# Autodesk Inventor assembly: Ensemble1
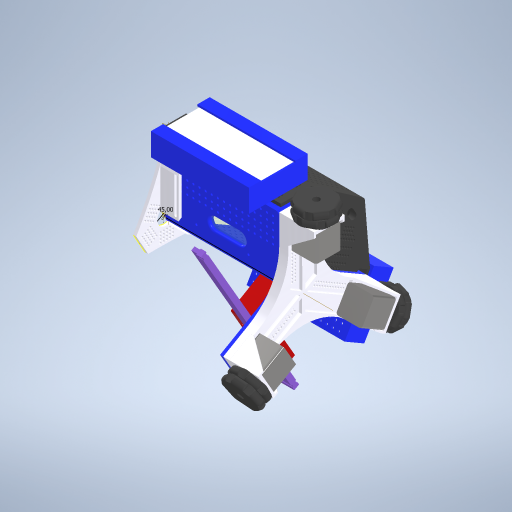
[picture p0: Inventor's stored thumbnail of the model, 512x512]
Saved by Autodesk Inventor 2024.1 (Build 281209000, 209)
## iProperties
Created: 2024-04-28
Part Number: Ensemble1
Document SubType Name: Assembly
Designer: chass
Author: chass
## Documents named in this file (14)
- C:\Users\chass\Desktop\Poster_cdr\vue eclatee robot\Ensemble1.iam
- C:\Users\chass\Desktop\Poster_cdr\vue eclatee robot\embase_tricorps_1.0.ipt
- C:\Users\chass\Desktop\Poster_cdr\vue eclatee robot\arbre_d_attache (1).ipt
- C:\Users\chass\Desktop\Poster_cdr\vue eclatee robot\mur_extension_2.ipt
- C:\Users\chass\Desktop\Poster_cdr\vue eclatee robot\couvercle_3roues2.ipt
- C:\Users\chass\Desktop\Poster_cdr\vue eclatee robot\actionneur_Support2.ipt
- C:\Users\chass\Desktop\Poster_cdr\vue eclatee robot\actionneur_doigt.ipt
- C:\Users\chass\Desktop\Poster_cdr\vue eclatee robot\support batterie.ipt
- C:\Users\chass\Desktop\Poster_cdr\vue eclatee robot\BAU.ipt
- C:\Users\chass\Desktop\Poster_cdr\vue eclatee robot\batt.ipt
- C:\Users\chass\Desktop\Poster_cdr\vue eclatee robot\roue.ipt
- C:\Users\chass\Desktop\Poster_cdr\vue eclatee robot\servomoteur.ipt
- C:\Users\chass\Desktop\Poster_cdr\vue eclatee robot\moteur_pasApas.ipt
- C:\Users\chass\Desktop\Poster_cdr\vue eclatee robot\roue_actionneur.ipt
## Components (22 placed, 13 different names)
1. embase_tricorps_1.0:1 — Placage:1, Placage:2, Placage:20, Placage:21, Placage:24, Placage:25, Placage:28, Placage:29, Placage:34, Placage:35, Placage:36, Placage:37, Placage:38, Placage:39, Placage:40, Placage:41, Placage:42
2. arbre_d_attache (1):1 — Placage:1, Placage:2, Placage:3, Placage:4, Placage:5, Placage:6, Placage:9, Placage:10, Placage:11, Placage:12
3. mur_extension_2:1
4. couvercle_3roues2:1 — Placage:3, Placage:4, Placage:13
5. actionneur_Support2:1 — Placage:5, Placage:6, Placage:7, Placage:8, Placage:32, Placage:33
6. actionneur_doigt:1 — Placage:7, Placage:8
7. support batterie:1 — Placage:9, Placage:10, Placage:14, Placage:15, Placage:16
8. support batterie:2 — Placage:11, Placage:12, Placage:17, Placage:18, Placage:19
9. BAU:1 — Placage:13
10. batt:1 — Placage:17, Placage:18, Placage:19
11. batt:2 — Placage:14, Placage:15, Placage:16
12. roue:3 — Placage:20, Placage:21, Placage:22, Placage:23
13. roue:4 — Placage:22, Placage:23
14. roue:5 — Placage:26, Placage:27
15. roue:6 — Placage:24, Placage:25, Placage:26, Placage:27
16. roue:7 — Placage:30, Placage:31
17. roue:8 — Placage:28, Placage:29, Placage:30, Placage:31
18. servomoteur:1 — Placage:32, Placage:33, Placage:43
19. moteur_pasApas:1 — Placage:37, Placage:38, Placage:39
20. moteur_pasApas:2 — Placage:34, Placage:35, Placage:36
21. moteur_pasApas:3 — Placage:40, Placage:41, Placage:42
22. roue_actionneur:1 — Placage:43
## Relationships (43: Mate 43)
- Placage:1 [Mate]: embase_tricorps_1.0:1 ↔ arbre_d_attache (1):1
- Placage:2 [Mate]: embase_tricorps_1.0:1 ↔ arbre_d_attache (1):1
- Placage:3 [Mate]: arbre_d_attache (1):1 ↔ couvercle_3roues2:1
- Placage:4 [Mate]: arbre_d_attache (1):1 ↔ couvercle_3roues2:1
- Placage:5 [Mate]: arbre_d_attache (1):1 ↔ actionneur_Support2:1
- Placage:6 [Mate]: arbre_d_attache (1):1 ↔ actionneur_Support2:1
- Placage:7 [Mate]: actionneur_Support2:1 ↔ actionneur_doigt:1
- Placage:8 [Mate]: actionneur_Support2:1 ↔ actionneur_doigt:1
- Placage:9 [Mate]: arbre_d_attache (1):1 ↔ support batterie:1
- Placage:10 [Mate]: arbre_d_attache (1):1 ↔ support batterie:1
- Placage:11 [Mate]: arbre_d_attache (1):1 ↔ support batterie:2
- Placage:12 [Mate]: arbre_d_attache (1):1 ↔ support batterie:2
- Placage:13 [Mate]: couvercle_3roues2:1 ↔ BAU:1
- Placage:14 [Mate]: support batterie:1 ↔ batt:2
- Placage:15 [Mate]: support batterie:1 ↔ batt:2
- Placage:16 [Mate]: support batterie:1 ↔ batt:2
- Placage:17 [Mate]: support batterie:2 ↔ batt:1
- Placage:18 [Mate]: support batterie:2 ↔ batt:1
- Placage:19 [Mate]: support batterie:2 ↔ batt:1
- Placage:20 [Mate]: embase_tricorps_1.0:1 ↔ roue:3
- Placage:21 [Mate]: embase_tricorps_1.0:1 ↔ roue:3
- Placage:22 [Mate]: roue:3 ↔ roue:4
- Placage:23 [Mate]: roue:3 ↔ roue:4
- Placage:24 [Mate]: embase_tricorps_1.0:1 ↔ roue:6
- Placage:25 [Mate]: embase_tricorps_1.0:1 ↔ roue:6
- Placage:26 [Mate]: roue:5 ↔ roue:6
- Placage:27 [Mate]: roue:5 ↔ roue:6
- Placage:28 [Mate]: embase_tricorps_1.0:1 ↔ roue:8
- Placage:29 [Mate]: embase_tricorps_1.0:1 ↔ roue:8
- Placage:30 [Mate]: roue:7 ↔ roue:8
- Placage:31 [Mate]: roue:7 ↔ roue:8
- Placage:32 [Mate]: actionneur_Support2:1 ↔ servomoteur:1
- Placage:33 [Mate]: actionneur_Support2:1 ↔ servomoteur:1
- Placage:34 [Mate]: embase_tricorps_1.0:1 ↔ moteur_pasApas:2
- Placage:35 [Mate]: embase_tricorps_1.0:1 ↔ moteur_pasApas:2
- Placage:36 [Mate]: embase_tricorps_1.0:1 ↔ moteur_pasApas:2
- Placage:37 [Mate]: embase_tricorps_1.0:1 ↔ moteur_pasApas:1
- Placage:38 [Mate]: embase_tricorps_1.0:1 ↔ moteur_pasApas:1
- Placage:39 [Mate]: embase_tricorps_1.0:1 ↔ moteur_pasApas:1
- Placage:40 [Mate]: embase_tricorps_1.0:1 ↔ moteur_pasApas:3
- Placage:41 [Mate]: embase_tricorps_1.0:1 ↔ moteur_pasApas:3
- Placage:42 [Mate]: embase_tricorps_1.0:1 ↔ moteur_pasApas:3
- Placage:43 [Mate]: servomoteur:1 ↔ roue_actionneur:1
